# Autodesk Inventor assembly: A_hermes
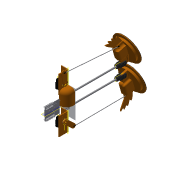
[picture p0: Inventor's stored thumbnail of the model, 180x180]
Saved by Autodesk Inventor 2016 (Build 200138000, 138)
## iProperties
Created: 2016-02-23
Part Number: A_hermes
Document SubType Name: Assembly
Designer: Mateusz
Author: Mateusz
## Documents named in this file (14)
- D:\PROJECTS\2016_biped\hermes\mechanics_tmp\A_hermes.iam
- D:\PROJECTS\2016_biped\hermes\mechanics_tmp\L1_legs_001.ipt
- D:\PROJECTS\2016_biped\hermes\mechanics_tmp\L2_foot_001.ipt
- D:\PROJECTS\2016_biped\hermes\mechanics_tmp\L3_ankle_001.ipt
- D:\PROJECTS\2016_biped\hermes\mechanics_tmp\P_threaded_rod_001.ipt
- D:\PROJECTS\2016_biped\hermes\mechanics_tmp\P_sole_001.ipt
- D:\PROJECTS\2016_biped\hermes\mechanics_tmp\P_foot_001.ipt
- D:\PROJECTS\2016_biped\hermes\mechanics_tmp\A_ankle_wing_001.iam
- D:\PROJECTS\2016_biped\hermes\mechanics_tmp\GEFM_10_1.ipt
- D:\PROJECTS\2016_biped\hermes\mechanics_tmp\GERM_10_F_2.ipt
- D:\PROJECTS\2016_biped\hermes\mechanics_tmp\P_bearing_fi10.ipt
- D:\PROJECTS\2016_biped\hermes\mechanics_tmp\A_hips_001.iam
- D:\PROJECTS\2016_biped\hermes\mechanics_tmp\A_snap_001.iam
- D:\PROJECTS\2016_biped\hermes\mechanics_tmp\A_ankle_wing_001_MIR.iam
## Components (22 placed, 13 different names)
1. L1_legs_001:1 — Mate:1, Mate:2, Mate:3, Mate:4, Mate:5, Flush:1, Mate:6, Mate:11, Mate:12, Mate:32, Mate:43, Mate:44
2. L2_foot_001:1 — Mate:7, Mate:8, Flush:4, Mate:15, Mate:18
3. L3_ankle_001:1 — Mate:4, Mate:5, Mate:7, Mate:8, Mate:27, Angle:1, Mate:28, Mate:33, Mate:41
4. L2_foot_001:2 — Mate:9, Mate:10
5. L3_ankle_001:2 — Flush:1, Mate:6, Mate:9, Mate:10, Mate:42, Flush:8, Mate:46, Flush:10
6. P_threaded_rod_001:1 — Mate:11, Insert:2
7. P_threaded_rod_001:2 — Mate:12, Mate:37, Insert:4
8. A_hips_001:1 [sub-assembly] — Mate:34, Flush:7, Mate:35, Mate:36, Mate:37, Mate:47
9. P_sole_001:1 — Flush:4, Mate:15, Flush:5
10. P_foot_001:1 — Flush:5, Mate:18, Insert:1
11. A_ankle_wing_001:1 [sub-assembly] — Mate:27, Angle:1, Mate:28, Insert:1, Mate:38
12. GEFM_10_1:1 — Mate:29, Mate:30, Mate:31, Mate:33
13. GERM_10_F_2:1 — Mate:29, Insert:2, Mate:30, Flush:6, Mate:32
14. P_bearing_fi10:1 — Flush:6, Mate:31
15. A_snap_001:1 [sub-assembly] — Mate:35, Mate:36, Mate:38
16. GEFM_10_1:2
17. GERM_10_F_2:2 — Insert:3, Insert:4, Mate:41
18. P_bearing_fi10:2 — Insert:3, Mate:44
19. A_ankle_wing_001_MIR:1 [sub-assembly] — Mate:42, Flush:8, Mate:43, Mate:48, Insert:5
20. P_sole_001:3 — Mate:45, Flush:10
21. P_foot_001:3 — Mate:45, Mate:46
22. A_snap_001:2 [sub-assembly] — Mate:47, Mate:48, Insert:5
## Relationships (50: Mate 36, Flush 8, Insert 5, Angle 1)
- Mate:1: L1_legs_001:1
- Mate:2: L1_legs_001:1
- Mate:3: L1_legs_001:1
- Mate:4: L1_legs_001:1 ↔ L3_ankle_001:1
- Mate:5: L1_legs_001:1 ↔ L3_ankle_001:1
- Flush:1: L1_legs_001:1 ↔ L3_ankle_001:2
- Mate:6: L1_legs_001:1 ↔ L3_ankle_001:2
- Mate:7: L2_foot_001:1 ↔ L3_ankle_001:1
- Mate:8: L2_foot_001:1 ↔ L3_ankle_001:1
- Mate:9: L2_foot_001:2 ↔ L3_ankle_001:2
- Mate:10: L2_foot_001:2 ↔ L3_ankle_001:2
- Mate:11: L1_legs_001:1 ↔ P_threaded_rod_001:1
- Mate:12: L1_legs_001:1 ↔ P_threaded_rod_001:2
- Flush:4: L2_foot_001:1 ↔ P_sole_001:1
- Mate:15: L2_foot_001:1 ↔ P_sole_001:1
- Flush:5: P_sole_001:1 ↔ P_foot_001:1
- Mate:18: L2_foot_001:1 ↔ P_foot_001:1
- Mate:27: L3_ankle_001:1 ↔ A_ankle_wing_001:1
- Angle:1 (0 deg): L3_ankle_001:1 ↔ A_ankle_wing_001:1
- Mate:28: L3_ankle_001:1 ↔ A_ankle_wing_001:1
- Insert:1: P_foot_001:1 ↔ A_ankle_wing_001:1
- Mate:29: GEFM_10_1:1 ↔ GERM_10_F_2:1
- Insert:2: P_threaded_rod_001:1 ↔ GERM_10_F_2:1
- Mate:30: GEFM_10_1:1 ↔ GERM_10_F_2:1
- Flush:6: GERM_10_F_2:1 ↔ P_bearing_fi10:1
- Mate:31: GEFM_10_1:1 ↔ P_bearing_fi10:1
- Mate:32: L1_legs_001:1 ↔ GERM_10_F_2:1
- Mate:33: L3_ankle_001:1 ↔ GEFM_10_1:1
- Mate:34: A_hips_001:1
- Flush:7: A_hips_001:1
- Mate:35: A_hips_001:1 ↔ A_snap_001:1
- Mate:36: A_hips_001:1 ↔ A_snap_001:1
- Mate:37: P_threaded_rod_001:2 ↔ A_hips_001:1
- Mate:38: A_ankle_wing_001:1 ↔ A_snap_001:1
- [Mate]: GEFM_10_1:2 ↔ GERM_10_F_2:2
- [Mate]: GEFM_10_1:2 ↔ GERM_10_F_2:2
- Insert:3: GERM_10_F_2:2 ↔ P_bearing_fi10:2
- Insert:4: P_threaded_rod_001:2 ↔ GERM_10_F_2:2
- Mate:41: L3_ankle_001:1 ↔ GERM_10_F_2:2
- Mate:42: L3_ankle_001:2 ↔ A_ankle_wing_001_MIR:1
- Flush:8: L3_ankle_001:2 ↔ A_ankle_wing_001_MIR:1
- Mate:43: L1_legs_001:1 ↔ A_ankle_wing_001_MIR:1
- Mate:44: L1_legs_001:1 ↔ P_bearing_fi10:2
- [Flush]: P_sole_001:3 ↔ P_foot_001:3
- Mate:45: P_sole_001:3 ↔ P_foot_001:3
- Mate:46: L3_ankle_001:2 ↔ P_foot_001:3
- Flush:10: L3_ankle_001:2 ↔ P_sole_001:3
- Mate:47: A_hips_001:1 ↔ A_snap_001:2
- Mate:48: A_ankle_wing_001_MIR:1 ↔ A_snap_001:2
- Insert:5: A_ankle_wing_001_MIR:1 ↔ A_snap_001:2
## Named parameters: d63_d49 = 0 mm, d64_d51 = 0 mm, d73_d29 = 0 mm
